# Autodesk Inventor assembly: PWTR-0050
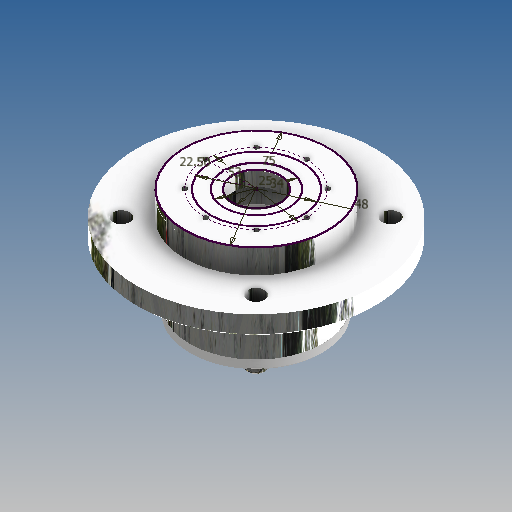
[picture p0: Inventor's stored thumbnail of the model, 512x512]
Saved by Autodesk Inventor 2021.1 (Build 251245000, 245)
## iProperties
Created: 2020-08-27
Part Number: PWTR-0050
Document SubType Name: Assembly
Designer: alid
Description: Transfer Box Lower Shaft Bonnet
Author: alid
Revision Number: A
## Documents named in this file (7)
- C:\Vault Workspace\Design Data\Projects\PRJ0095\PWTR-CTO\PWTR-0050.iam
- C:\Vault Workspace\Design Data\Projects\PRJ0095\PWTR-CTO\PWTR-0046.ipt
- C:\Vault Workspace\Design Data\Projects\PRJ0095\PWTR-CTO\PWTR-0047.ipt
- C:\Vault Workspace\Design Data\Projects\PRJ0095\PWTR-CTO\PWTR-0048.ipt
- C:\Vault Workspace\Design Data\Projects\PRJ0095\PWTR-CTO\PWTR-0051.ipt
- C:\Vault Workspace\Design Data\Projects\PRJ0095\PWTR-CTO\PWTR-0053.ipt
- C:\Vault Workspace\Design Data\Projects\PRJ0095\PWTR-CTO\PWTR-0060.ipt
## Components (10 placed, 6 different names)
1. PWTR-0046:1 — Rigid:1, Insert:4, Rotational:1
2. PWTR-0047:1
3. PWTR-0048:1
4. PWTR-0051:2 — Rigid:1, Insert:3
5. PWTR-0047:2 — Insert:4
6. PWTR-0060:1 — Rotational:1
7. PWTR-0053:1 — Insert:3
8. PWTR-0053:2
9. PWTR-0053:3
10. PWTR-0053:4
## Component patterns: (4 elements, first: PWTR-0053:1)
## Relationships (6: Insert 4, WeldJoint 1, RevoluteJoint 1)
- [Insert]: PWTR-0047:1 ↔ PWTR-0048:1
- [Insert]: PWTR-0046:1 ↔ PWTR-0047:1
- Rigid:1 [WeldJoint]: PWTR-0046:1 ↔ PWTR-0051:2
- Insert:3: PWTR-0051:2 ↔ PWTR-0053:1
- Insert:4: PWTR-0046:1 ↔ PWTR-0047:2
- Rotational:1 [RevoluteJoint]: PWTR-0046:1 ↔ PWTR-0060:1
